# Autodesk Inventor assembly: SSEB-MX10-55
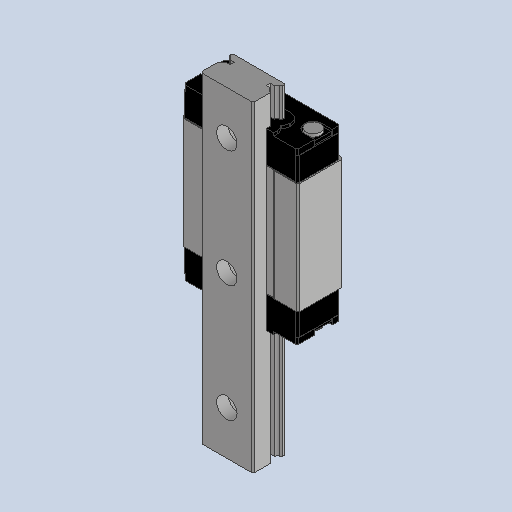
[picture p0: Inventor's stored thumbnail of the model, 512x512]
Saved by Autodesk Inventor 2025.2 (Build 292293000, 293)
## iProperties
Category: PARTsolutions
Company: MISUMI
Created: 2025-03-30
Part Number: SSEB-MX10-55
Catalog Web Link: www.cadenas.de
Description: SSEB, SSEB-MX, SSE2B, SSE2B-MX, RSEB, RSE2B-Miniature Linear Guides Standard Blocks/Light Preload High Grade-L Selectable Type
Vendor: MISUMI
Document SubType Name: Assembly
Designer: psAdmin
Manufacturer: MISUMI
Mass: 5.67328 g
Surface Area: 44.6536 cm^2
Volume: 5.67328 cm^3
Density: 1 g/cm^3
PSOL_IDENT_0: {$CADENAS_DATA/23d-libs/misumi/metric/06_linear_guides/re2b_asmtab.prj},261 {VTYP=3D},{STYP=ASSTAB},
PSOL_IDENT_1: {NB=SSEB-MX10-55},{LINA=SSEB-MX10-55},{NN=SSEB, SSEB-MX, SSE2B, SSE2B-MX, RSEB, RSE2B},{DATE=04.04.2
PSOL_IDENT_2: 024 07:12:35},{GEOMDATE=07.03.2024 00:33:43},{VERSION=},{LINEID=160},{WBVAR=ST,MAT,MX,NOB,GREASE,LS,
PSOL_IDENT_3: ALT1,ALT2,ALT3,ALT4},{WBNUMERIC=LS}  {NB=SSEB-MX10-55},{LINA=SSEB-MX10-55},{KT=DUMMY},{PN=SSEB-MX10-
PSOL_IDENT_4: 55},{RT=B},{TYPE=SSEB},{ST=S},{MAT=S},{MX=-MX},{MXALG='', 'w/o MX(Lubrication unit)', '-MX', 'with M
PSOL_IDENT_5: X(Lubrication unit)'},{NOB=},{H=10},{GREASE=},{GREASEALG='','Normal'},{LT=Selectable},{LS=55},{HARD=
PSOL_IDENT_6: 56HRC~},{W=20},{L1=30.0},{B=15},{C=10},{SLL=M3x3},{L2=19.0},{K=7.8},{CBB=0.3},{W1=9},{W2=5.5},{H1=5.
PSOL_IDENT_7: 5},{CAA=0.3},{DD1DD2HH=3.5x6x3.5},{F=20},{G=7.5},{ALT1=},{ALT1ALG= '', 'w/o MC (Tapped Holes)', '-MC'
PSOL_IDENT_8: , 'with MC (Tapped Holes)' },{MC=M4},{ALT2=},{ALT2L=2.5},{ALT2N=5},{M=3},{LL=},{L0=35,55,75,95,115,1
PSOL_IDENT_9: 35,155,175,195,215,235,255,275,295,315,335,355,355,375,395,415,435,455,475,495,515,535,555,575,595,6
PSOL_IDENT_10: 15,635},{REC1=   '','w/o Rail Ends Cut alteration','-LLC','with LLC (Left End Cut)','-RLC','with RLC
PSOL_IDENT_11: (Right End Cut)','-LLC-RLC','with Both End Cut'   },{ST1='S', 'w/o Surface Treatment','R','Low Temp
PSOL_IDENT_12: erature Black Chrome Plating'},{MAT2='S','Stainless Steel'},{ALT3=},{ALT3ALG= '' , 'w/o WC (Pair of
PSOL_IDENT_13: Rails)' , '-WC' , 'with WC (Set Pair of Rails)' },{ALT4=},{ALT4ALG= '','Not applicable' },{PPATH=seb
PSOL_IDENT_14: _series/seb_asmtpl.prj}
NB: SSEB-MX10-55
NN: SSEB, SSEB-MX, SSE2B, SSE2B-MX, RSEB, RSE2B
NT: Miniature Linear Guides Standard Blocks/Light Preload High Grade-L Selectable Type
NBSYN: $PN.
LINA: SSEB-MX10-55
CATALOG: Misumi
PN: SSEB-MX10-55
ST: w/o Surface Treatment
MAT: Stainless Steel
MX: with MX(Lubrication unit)
NOB: 1
H: 10
GREASE: Normal
LS: 55
W: 20
L1: 30
B: 15
C: 10
SLL: M3x3
L2: 19
K: 7.8
CBB: 0.3
W1: 9
W2: 5.5
H1: 5.5
CAA: 0.3
DD1DD2HH: 3.5x6x3.5
F: 20
G: 7.5
ALT1: w/o MC (Tapped Holes)
ALT2: w/o Rail Ends Cut alteration
ALT3: w/o WC (Pair of Rails)
ALT4: Not applicable
SUPPLIER: MISUMI
ARTICLENO: SSEB-MX10-55
BOMINFO: SSEB-MX10-55
CREATOR: CADENAS GmbH
Title: SSEB-MX10-55
Author: Cadenas PARTsolutions
Comments: Miniature Linear Guides Standard Blocks/Light Preload High Grade-L Selectable Type
## Documents named in this file (3)
- C:\Users\haruy\Documents\ロボコン\NHK2025\cad\nagahisa\odom\SSEB-MX10-55.iam
- C:\Users\haruy\Documents\ロボコン\NHK2025\cad\nagahisa\odom\SSEB-MX10-55_r.ipt
- C:\Users\haruy\Documents\ロボコン\NHK2025\cad\nagahisa\odom\SSEB-MX10_b.ipt
## Components (2 placed, 2 different names)
1. SSEB-MX10-55_r:1 — to_block_Z@1 <-> to_rail_Z@2, to_block_YZ@1 <-> to_rail_YZ@2, フラッシュ:1
2. SSEB-MX10_b:1 — to_block_Z@1 <-> to_rail_Z@2, to_block_YZ@1 <-> to_rail_YZ@2, フラッシュ:1
## Relationships (3: Mate 1, Angle 1, Flush 1)
- to_block_Z@1 <-> to_rail_Z@2 [Mate]: SSEB-MX10-55_r:1 ↔ SSEB-MX10_b:1
- to_block_YZ@1 <-> to_rail_YZ@2 [Angle] (0 deg): SSEB-MX10-55_r:1 ↔ SSEB-MX10_b:1
- フラッシュ:1 [Flush] (5 mm): SSEB-MX10-55_r:1 ↔ SSEB-MX10_b:1
